# Autodesk Inventor assembly: Smaller Re-Entrant Flange
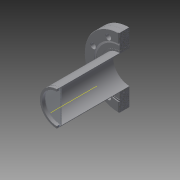
[picture p0: Inventor's stored thumbnail of the model, 180x180]
Saved by Autodesk Inventor 2015 (Build 190159000, 159)
## iProperties
Created: 2014-07-10
Part Number: Smaller Re-Entrant Flange
Document SubType Name: Assembly
Designer: I Rabey
Author: I Rabey
## Documents named in this file (6)
- C:\ColdMatter\CADFiles\EDM Machine\Microwave Detection Region\Re-entrant Flange\Smaller Version\Smaller Re-Entrant Flange.iam
- C:\ColdMatter\CADFiles\EDM Machine\Microwave Detection Region\Re-entrant Flange\Smaller Version\DN63CF Counter Bored.ipt
- C:\ColdMatter\CADFiles\EDM Machine\Microwave Detection Region\Re-entrant Flange\Smaller Version\Smaller Vacuum Cylinder.ipt
- C:\ColdMatter\CADFiles\EDM Machine\Microwave Detection Region\Re-entrant Flange\Smaller Version\Small Window.ipt
- C:\ColdMatter\CADFiles\EDM Machine\Microwave Detection Region\Re-entrant Flange\Smaller Version\Smaller Cap.ipt
- C:\ColdMatter\CADFiles\EDM Machine\Microwave Detection Region\Re-entrant Flange\Smaller Version\O-VO33.ipt
## Components (5 placed, 5 different names)
1. DN63CF Counter Bored:1 — Mate:1, Mate:2, Mate:3, Mate:4
2. Smaller Vacuum Cylinder:1 — Mate:3, Mate:4, Mate:5, Mate:6, Mate:9, Mate:10
3. Small Window:1 — Mate:5, Mate:6
4. Smaller Cap:1 — Mate:7, Mate:8, Mate:9, Mate:10, Mate:11
5. O-VO33:1 — Mate:7, Mate:8, Mate:11
## Relationships (11: Mate 11)
- Mate:1: DN63CF Counter Bored:1
- Mate:2: DN63CF Counter Bored:1
- Mate:3: DN63CF Counter Bored:1 ↔ Smaller Vacuum Cylinder:1
- Mate:4: DN63CF Counter Bored:1 ↔ Smaller Vacuum Cylinder:1
- Mate:5: Smaller Vacuum Cylinder:1 ↔ Small Window:1
- Mate:6: Smaller Vacuum Cylinder:1 ↔ Small Window:1
- Mate:7: Smaller Cap:1 ↔ O-VO33:1
- Mate:8: Smaller Cap:1 ↔ O-VO33:1
- Mate:9: Smaller Vacuum Cylinder:1 ↔ Smaller Cap:1
- Mate:10: Smaller Vacuum Cylinder:1 ↔ Smaller Cap:1
- Mate:11: Smaller Cap:1 ↔ O-VO33:1
